# Autodesk Inventor assembly: Motor-Pump cw
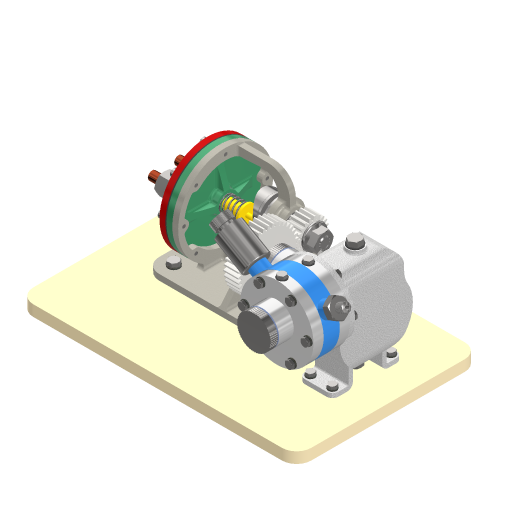
[picture p0: Inventor's stored thumbnail of the model, 512x512]
Saved by Autodesk Inventor 2024.2 (Build 282272000, 272)
## iProperties
Created: 2025-06-19
Part Number: Motor-Pump cw
Document SubType Name: Assembly
Designer: cw
Author: cw
## Documents named in this file (12)
- C:\zWSA2025 TP05 M1\Solution\Motor-Pump CW.iam
- C:\zWSA2025 TP05 M1\Solution\Table Top.ipt
- C:\zWSA2025 TP05 M1\Solution\Diaphragrm Pump.iam
- C:\zWSA2025 TP05 M1\Solution\Content Center\en-US\DIN 6885-1 A\DIN 6885 - A 5 x 5 x 18.ipt
- C:\zWSA2025 TP05 M1\Solution\Motor CW.iam
- C:\zWSA2025 TP05 M1\Solution\Spacer B005.ipt
- C:\zWSA2025 TP05 M1\Solution\Design Accelerator\Spur Gears1.iam
- C:\zWSA2025 TP05 M1\Solution\Content Center\en-US\ISO 4161\ISO 4161 - M16(1).ipt
- C:\zWSA2025 TP05 M1\Solution\Content Center\en-US\ISO 4017(1)\ISO 4017 - M6 x 16 - ISO.ipt
- C:\zWSA2025 TP05 M1\Solution\Content Center\en-US\ISO 7091\ISO 7091 - ST 6 - 100 HV.ipt
- C:\zWSA2025 TP05 M1\Solution\Content Center\en-US\ISO 4017(1)\ISO 4017 - M8 x 16 - ISO.ipt
- C:\zWSA2025 TP05 M1\Solution\Content Center\en-US\ISO 7091\ISO 7091 - ST 8 - 100 HV.ipt
## Components (25 placed, 11 different names)
1. Table Top:1 — Mate:1, Mate:2, Mate:3, Mate:4, Mate:5, Mate:6, Mate:27, Angle:1, Mate:31, Angle:2
2. Motor CW:1 [sub-assembly] — Mate:1, Mate:2, Mate:3, Mate:7, Mate:8, Mate:9, Rotation:1(FullMotionCheck), Mate:15, Mate:16, Mate:19, Mate:21, Flush:1, Mate:28
3. Diaphragrm Pump:1 [sub-assembly] — Mate:4, Mate:5, Mate:6, Mate:10, Mate:11, Mate:12, Rotation:1(FullMotionCheck), Mate:13, Mate:14, Mate:17, Mate:18, Mate:22, Mate:24, Flush:2, Mate:32
4. DIN 6885-1 A A 5 x 5 x 18:1 — Mate:7, Mate:8, Mate:9
5. DIN 6885-1 A A 5 x 5 x 18:2 — Mate:10, Mate:11, Mate:12
6. Spacer B005:1 — Mate:13, Mate:14
7. Spur Gears:1 [sub-assembly] — Mate:15, Mate:16, Mate:17, Mate:18, Mate:20, Mate:23, Flush:1, Flush:2
8. ISO 4161 M16:1 — Mate:19, Mate:20, Mate:21
9. ISO 4161 M16:2 — Mate:22, Mate:23, Mate:24
10. ISO 4017 M6 x 16:1 — Mate:25, Mate:26, Mate:27, Angle:1
11. ISO 7091 ST 6 - 100 HV:1 — Mate:25, Mate:26, Mate:28
12. ISO 4017 M6 x 16:2
13. ISO 7091 ST 6 - 100 HV:2
14. ISO 4017 M6 x 16:3
15. ISO 7091 ST 6 - 100 HV:3
16. ISO 4017 M6 x 16:4
17. ISO 7091 ST 6 - 100 HV:4
18. ISO 4017 M8 x 16:1 — Mate:29, Mate:30, Mate:31, Angle:2
19. ISO 7091 ST 8 - 100 HV:1 — Mate:29, Mate:30, Mate:32
20. ISO 4017 M8 x 16:2
21. ISO 7091 ST 8 - 100 HV:2
22. ISO 4017 M8 x 16:3
23. ISO 7091 ST 8 - 100 HV:3
24. ISO 4017 M8 x 16:4
25. ISO 7091 ST 8 - 100 HV:4
## Component patterns: (4 elements, first: ISO 4017 M6 x 16:1 + ISO 7091 ST 6 - 100 HV:1), (4 elements, first: ISO 4017 M8 x 16:1 + ISO 7091 ST 8 - 100 HV:1)
## Relationships (37: Mate 32, Flush 2, Angle 2, RelateRotation 1)
- Mate:1: Table Top:1 ↔ Motor CW:1
- Mate:2: Table Top:1 ↔ Motor CW:1
- Mate:3: Table Top:1 ↔ Motor CW:1
- Mate:4: Table Top:1 ↔ Diaphragrm Pump:1
- Mate:5: Table Top:1 ↔ Diaphragrm Pump:1
- Mate:6: Table Top:1 ↔ Diaphragrm Pump:1
- Mate:7: Motor CW:1 ↔ DIN 6885-1 A A 5 x 5 x 18:1
- Mate:8: Motor CW:1 ↔ DIN 6885-1 A A 5 x 5 x 18:1
- Mate:9: Motor CW:1 ↔ DIN 6885-1 A A 5 x 5 x 18:1
- Mate:10: Diaphragrm Pump:1 ↔ DIN 6885-1 A A 5 x 5 x 18:2
- Mate:11: Diaphragrm Pump:1 ↔ DIN 6885-1 A A 5 x 5 x 18:2
- Mate:12: Diaphragrm Pump:1 ↔ DIN 6885-1 A A 5 x 5 x 18:2
- Rotation:1(FullMotionCheck) [RelateRotation]: Motor CW:1 ↔ Diaphragrm Pump:1
- Mate:13: Diaphragrm Pump:1 ↔ Spacer B005:1
- Mate:14: Diaphragrm Pump:1 ↔ Spacer B005:1
- Mate:15: Motor CW:1 ↔ Spur Gears:1
- Mate:16: Motor CW:1 ↔ Spur Gears:1
- Mate:17: Diaphragrm Pump:1 ↔ Spur Gears:1
- Mate:18: Diaphragrm Pump:1 ↔ Spur Gears:1
- Mate:19: Motor CW:1 ↔ ISO 4161 M16:1
- Mate:20: Spur Gears:1 ↔ ISO 4161 M16:1
- Mate:21: Motor CW:1 ↔ ISO 4161 M16:1
- Mate:22: Diaphragrm Pump:1 ↔ ISO 4161 M16:2
- Mate:23: Spur Gears:1 ↔ ISO 4161 M16:2
- Mate:24: Diaphragrm Pump:1 ↔ ISO 4161 M16:2
- Flush:1: Motor CW:1 ↔ Spur Gears:1
- Flush:2: Diaphragrm Pump:1 ↔ Spur Gears:1
- Mate:25: ISO 4017 M6 x 16:1 ↔ ISO 7091 ST 6 - 100 HV:1
- Mate:26: ISO 4017 M6 x 16:1 ↔ ISO 7091 ST 6 - 100 HV:1
- Mate:27: Table Top:1 ↔ ISO 4017 M6 x 16:1
- Mate:28: Motor CW:1 ↔ ISO 7091 ST 6 - 100 HV:1
- Angle:1 (0 deg): Table Top:1 ↔ ISO 4017 M6 x 16:1
- Mate:29: ISO 4017 M8 x 16:1 ↔ ISO 7091 ST 8 - 100 HV:1
- Mate:30: ISO 4017 M8 x 16:1 ↔ ISO 7091 ST 8 - 100 HV:1
- Mate:31: Table Top:1 ↔ ISO 4017 M8 x 16:1
- Mate:32: Diaphragrm Pump:1 ↔ ISO 7091 ST 8 - 100 HV:1
- Angle:2 (0 deg): Table Top:1 ↔ ISO 4017 M8 x 16:1
